# Autodesk Inventor assembly: Remote
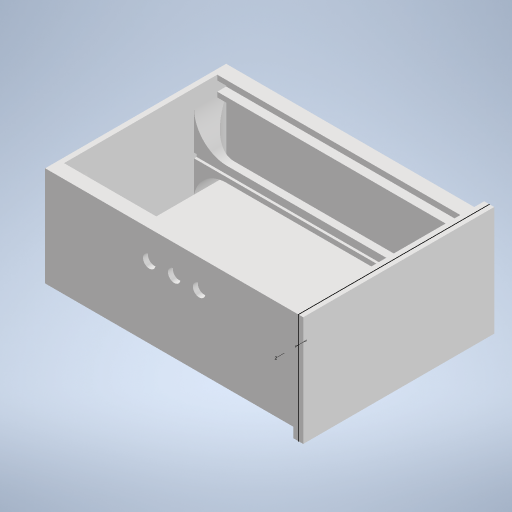
[picture p0: Inventor's stored thumbnail of the model, 512x512]
Saved by Autodesk Inventor 2023 (Build 270158000, 158)
## iProperties
Created: 2023-03-27
Part Number: Remote
Document SubType Name: Assembly
Designer: eleves
Author: eleves
## Documents named in this file (3)
- C:\Users\eleves\Desktop\PE-SM\3D\Remote.iam
- C:\Users\eleves\Desktop\PE-SM\3D\Remote.ipt
- C:\Users\eleves\Desktop\PE-SM\3D\Cache_remote.ipt
## Components (2 placed, 2 different names)
1. Remote:1 — Affleurement:1
2. Cache_remote:1 — Affleurement:1
## Relationships (1: Flush 1)
- Affleurement:1 [Flush]: Remote:1 ↔ Cache_remote:1
